# Autodesk Inventor assembly: Scananlage_Adrian
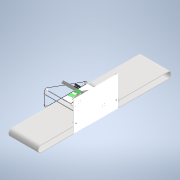
[picture p0: Inventor's stored thumbnail of the model, 180x180]
Saved by Autodesk Inventor 2021 (Build 250183000, 183)
## iProperties
Created: 2022-07-12
Part Number: Scananlage_Adrian
Document SubType Name: Assembly
Designer: adria
Mass: 34959.8 g
Surface Area: 77259.1 cm^2
Volume: 43992.2 cm^3
Density: 0.794683 g/cm^3
Author: adria
## Documents named in this file (16)
- C:\Users\adria\OneDrive - tum.de\G2_Waste-Recycling\CAD\Scananlage_Adrian.iam
- C:\Users\adria\OneDrive - tum.de\G2_Waste-Recycling\CAD\Adrian_Box.iam
- C:\Users\adria\OneDrive - tum.de\G2_Waste-Recycling\CAD\Adrian_Stangeantrieb.iam
- C:\Users\adria\OneDrive - tum.de\G2_Waste-Recycling\CAD\Adrian_Rolle.iam
- C:\Users\adria\OneDrive - tum.de\G2_Waste-Recycling\CAD\stepper-motor-nema17-simplified-model-1.snapshot.3\motor.ipt
- C:\Users\adria\OneDrive - tum.de\G2_Waste-Recycling\CAD\Adrian_Drehteller.iam
- C:\Users\adria\OneDrive - tum.de\G2_Waste-Recycling\CAD\Adrian_Cameraarm.iam
- C:\Users\adria\OneDrive - tum.de\G2_Waste-Recycling\CAD\Adrian_Faden.ipt
- C:\Users\adria\OneDrive - tum.de\G2_Waste-Recycling\CAD\Stange_SCHIEBER.ipt
- C:\Users\adria\OneDrive - tum.de\G2_Waste-Recycling\CAD\GT2 Timing Pulley T40.ipt
- C:\Users\adria\OneDrive - tum.de\G2_Waste-Recycling\CAD\Adrian_Riemen.ipt
- C:\Users\adria\OneDrive - tum.de\G2_Waste-Recycling\CAD\Assembly Raspberry Pi 4 Model B step.ipt
- C:\Users\adria\OneDrive - tum.de\G2_Waste-Recycling\CAD\Ethernet SmoothStepper_ASSEMBLY.ipt
- C:\Users\adria\Documents\Inventor\Content Center Files\R2021\de-DE\ISO 1207(2)\ISO 1207 - M2 x 6.ipt
- C:\Users\adria\Documents\Inventor\Content Center Files\R2021\de-DE\ISO 4762(2)\ISO 4762 - M3 x 30ISO.ipt
- C:\Users\adria\OneDrive - tum.de\G2_Waste-Recycling\CAD\Adrian_Förderband.ipt
## Components (35 placed, 15 different names)
1. Adrian_Box:1 [sub-assembly] — Passend:1, Fluchtend:1, Passend:2, Passend:3, Passend:4, Passend:5, Passend:6, Passend:7, Passend:8, Passend:9, Passend:10, Passend:11, Passend:12, Passend:13, Passend:14, Passend:15, Passend:16, Passend:17, Passend:18, Passend:19, Passend:24, Passend:25, Passend:32, Fluchtend:3, Passend:33, Passend:34, Fluchtend:4, Passend:44, Passend:45, Passend:46, Passend:47, Passend:48, Passend:49, Passend:50, Passend:51, Passend:52, Passend:53, Passend:54, Passend:55, Passend:56, Passend:57, Passend:58, Passend:59, Passend:60, Passend:61, Passend:62, Passend:63, Passend:64, Passend:65, Passend:66, Passend:67, Fluchtend:6, Fluchtend:7, Fluchtend:10
2. Adrian_Stangeantrieb:1 [sub-assembly] — Passend:1, Fluchtend:1, Passend:31
3. Adrian_Rolle:1 [sub-assembly] — Passend:2, Passend:3
4. Adrian_Rolle:2 [sub-assembly] — Passend:6, Passend:9, Passend:23
5. Adrian_Rolle:3 [sub-assembly] — Passend:5, Passend:8, Passend:22
6. Adrian_Rolle:4 [sub-assembly] — Passend:4, Passend:7, Passend:26, Passend:27
7. motor:1 — Passend:10, Passend:11, Passend:16, Passend:28, Passend:29, Winkel:1, Fluchtend:2
8. motor:3 — Passend:12, Passend:13, Passend:14, Passend:15, Passend:20, Passend:21
9. Adrian_Drehteller:1 [sub-assembly] — Passend:17, Passend:18, Passend:19
10. Adrian_Cameraarm:1 [sub-assembly] — Passend:20, Passend:21
11. Adrian_Faden:1 — Passend:22, Passend:24, Passend:27, Tangential:1
12. Adrian_Faden:2 — Passend:23, Passend:25
13. Stange_SCHIEBER:1 — Passend:26, Tangential:1
14. GT2 Timing Pulley T40:1 — Passend:28, Passend:29, Passend:30
15. Adrian_Riemen:1 — Winkel:1, Passend:30, Passend:31, Fluchtend:2
16. Assembly Raspberry Pi 4 Model B step:1 — Passend:32, Fluchtend:3, Passend:33, Passend:35, Passend:38, Passend:39, Passend:40, Passend:41
17. Ethernet SmoothStepper_ASSEMBLY:1 — Passend:34, Fluchtend:4, Passend:35, Passend:36, Passend:37, Passend:42, Passend:43
18. ISO 1207 M2 x 6:1 — Passend:37, Passend:43
19. ISO 1207 M2 x 6:2 — Passend:36, Passend:42
20. ISO 1207 M2 x 6:3 — Passend:39, Passend:40
21. ISO 1207 M2 x 6:4 — Passend:38, Passend:41
22. ISO 4762 M3 x 30:3 — Passend:46, Passend:49
23. ISO 4762 M3 x 30:4 — Passend:44, Passend:51
24. ISO 4762 M3 x 30:5 — Passend:47, Passend:50
25. ISO 4762 M3 x 30:6 — Passend:45, Passend:48
26. ISO 4762 M3 x 30:7 — Passend:52, Passend:58
27. ISO 4762 M3 x 30:8 — Passend:55, Passend:56
28. ISO 4762 M3 x 30:9 — Passend:53, Passend:59
29. ISO 4762 M3 x 30:10 — Passend:54, Passend:57
30. ISO 4762 M3 x 30:11 — Passend:61, Passend:65
31. ISO 4762 M3 x 30:12 — Passend:60, Passend:67
32. ISO 4762 M3 x 30:13 — Passend:63, Passend:64
33. ISO 4762 M3 x 30:14 — Passend:62, Passend:66
34. Adrian_Förderband:1 — Fluchtend:5, Fluchtend:6, Fluchtend:7, Fluchtend:8
35. Adrian_Förderband:2 — Fluchtend:5, Fluchtend:8
## Relationships (78: Mate 67, Flush 9, Tangent 1, Angle 1)
- Passend:1 [Mate]: Adrian_Box:1 ↔ Adrian_Stangeantrieb:1
- Fluchtend:1 [Flush]: Adrian_Box:1 ↔ Adrian_Stangeantrieb:1
- Passend:2 [Mate]: Adrian_Box:1 ↔ Adrian_Rolle:1
- Passend:3 [Mate]: Adrian_Box:1 ↔ Adrian_Rolle:1
- Passend:4 [Mate]: Adrian_Box:1 ↔ Adrian_Rolle:4
- Passend:5 [Mate]: Adrian_Box:1 ↔ Adrian_Rolle:3
- Passend:6 [Mate]: Adrian_Box:1 ↔ Adrian_Rolle:2
- Passend:7 [Mate]: Adrian_Box:1 ↔ Adrian_Rolle:4
- Passend:8 [Mate]: Adrian_Box:1 ↔ Adrian_Rolle:3
- Passend:9 [Mate]: Adrian_Box:1 ↔ Adrian_Rolle:2
- Passend:10 [Mate]: Adrian_Box:1 ↔ motor:1
- Passend:11 [Mate]: Adrian_Box:1 ↔ motor:1
- Passend:12 [Mate]: Adrian_Box:1 ↔ motor:3
- Passend:13 [Mate]: Adrian_Box:1 ↔ motor:3
- Passend:14 [Mate]: Adrian_Box:1 ↔ motor:3
- Passend:15 [Mate]: Adrian_Box:1 ↔ motor:3
- Passend:16 [Mate]: Adrian_Box:1 ↔ motor:1
- Passend:17 [Mate]: Adrian_Box:1 ↔ Adrian_Drehteller:1
- Passend:18 [Mate]: Adrian_Box:1 ↔ Adrian_Drehteller:1
- Passend:19 [Mate]: Adrian_Box:1 ↔ Adrian_Drehteller:1
- Passend:20 [Mate]: motor:3 ↔ Adrian_Cameraarm:1
- Passend:21 [Mate]: motor:3 ↔ Adrian_Cameraarm:1
- Passend:22 [Mate]: Adrian_Rolle:3 ↔ Adrian_Faden:1
- Passend:23 [Mate]: Adrian_Rolle:2 ↔ Adrian_Faden:2
- Passend:24 [Mate] (10 mm): Adrian_Box:1 ↔ Adrian_Faden:1
- Passend:25 [Mate] (10 mm): Adrian_Box:1 ↔ Adrian_Faden:2
- Passend:26 [Mate]: Adrian_Rolle:4 ↔ Stange_SCHIEBER:1
- Passend:27 [Mate]: Adrian_Rolle:4 ↔ Adrian_Faden:1
- Tangential:1: Adrian_Faden:1 ↔ Stange_SCHIEBER:1
- Passend:28 [Mate]: motor:1 ↔ GT2 Timing Pulley T40:1
- Passend:29 [Mate]: motor:1 ↔ GT2 Timing Pulley T40:1
- Winkel:1 [Angle] (0 deg): motor:1 ↔ Adrian_Riemen:1
- Passend:30 [Mate]: GT2 Timing Pulley T40:1 ↔ Adrian_Riemen:1
- Passend:31 [Mate]: Adrian_Stangeantrieb:1 ↔ Adrian_Riemen:1
- Fluchtend:2 [Flush] (-7 mm): motor:1 ↔ Adrian_Riemen:1
- Passend:32 [Mate]: Adrian_Box:1 ↔ Assembly Raspberry Pi 4 Model B step:1
- Fluchtend:3 [Flush] (40 mm): Adrian_Box:1 ↔ Assembly Raspberry Pi 4 Model B step:1
- Passend:33 [Mate] (40 mm): Adrian_Box:1 ↔ Assembly Raspberry Pi 4 Model B step:1
- Passend:34 [Mate]: Adrian_Box:1 ↔ Ethernet SmoothStepper_ASSEMBLY:1
- Fluchtend:4 [Flush] (40 mm): Adrian_Box:1 ↔ Ethernet SmoothStepper_ASSEMBLY:1
- Passend:35 [Mate] (40 mm): Assembly Raspberry Pi 4 Model B step:1 ↔ Ethernet SmoothStepper_ASSEMBLY:1
- Passend:36 [Mate]: Ethernet SmoothStepper_ASSEMBLY:1 ↔ ISO 1207 M2 x 6:2
- Passend:37 [Mate]: Ethernet SmoothStepper_ASSEMBLY:1 ↔ ISO 1207 M2 x 6:1
- Passend:38 [Mate]: Assembly Raspberry Pi 4 Model B step:1 ↔ ISO 1207 M2 x 6:4
- Passend:39 [Mate]: Assembly Raspberry Pi 4 Model B step:1 ↔ ISO 1207 M2 x 6:3
- Passend:40 [Mate]: Assembly Raspberry Pi 4 Model B step:1 ↔ ISO 1207 M2 x 6:3
- Passend:41 [Mate]: Assembly Raspberry Pi 4 Model B step:1 ↔ ISO 1207 M2 x 6:4
- Passend:42 [Mate]: Ethernet SmoothStepper_ASSEMBLY:1 ↔ ISO 1207 M2 x 6:2
- Passend:43 [Mate]: Ethernet SmoothStepper_ASSEMBLY:1 ↔ ISO 1207 M2 x 6:1
- Passend:44 [Mate]: Adrian_Box:1 ↔ ISO 4762 M3 x 30:4
- Passend:45 [Mate]: Adrian_Box:1 ↔ ISO 4762 M3 x 30:6
- Passend:46 [Mate]: Adrian_Box:1 ↔ ISO 4762 M3 x 30:3
- Passend:47 [Mate]: Adrian_Box:1 ↔ ISO 4762 M3 x 30:5
- Passend:48 [Mate]: Adrian_Box:1 ↔ ISO 4762 M3 x 30:6
- Passend:49 [Mate]: Adrian_Box:1 ↔ ISO 4762 M3 x 30:3
- Passend:50 [Mate]: Adrian_Box:1 ↔ ISO 4762 M3 x 30:5
- Passend:51 [Mate]: Adrian_Box:1 ↔ ISO 4762 M3 x 30:4
- Passend:52 [Mate]: Adrian_Box:1 ↔ ISO 4762 M3 x 30:7
- Passend:53 [Mate]: Adrian_Box:1 ↔ ISO 4762 M3 x 30:9
- Passend:54 [Mate]: Adrian_Box:1 ↔ ISO 4762 M3 x 30:10
- Passend:55 [Mate]: Adrian_Box:1 ↔ ISO 4762 M3 x 30:8
- Passend:56 [Mate]: Adrian_Box:1 ↔ ISO 4762 M3 x 30:8
- Passend:57 [Mate]: Adrian_Box:1 ↔ ISO 4762 M3 x 30:10
- Passend:58 [Mate]: Adrian_Box:1 ↔ ISO 4762 M3 x 30:7
- Passend:59 [Mate]: Adrian_Box:1 ↔ ISO 4762 M3 x 30:9
- Passend:60 [Mate]: Adrian_Box:1 ↔ ISO 4762 M3 x 30:12
- Passend:61 [Mate]: Adrian_Box:1 ↔ ISO 4762 M3 x 30:11
- Passend:62 [Mate]: Adrian_Box:1 ↔ ISO 4762 M3 x 30:14
- Passend:63 [Mate]: Adrian_Box:1 ↔ ISO 4762 M3 x 30:13
- Passend:64 [Mate]: Adrian_Box:1 ↔ ISO 4762 M3 x 30:13
- Passend:65 [Mate]: Adrian_Box:1 ↔ ISO 4762 M3 x 30:11
- Passend:66 [Mate]: Adrian_Box:1 ↔ ISO 4762 M3 x 30:14
- Passend:67 [Mate]: Adrian_Box:1 ↔ ISO 4762 M3 x 30:12
- Fluchtend:5 [Flush]: Adrian_Förderband:1 ↔ Adrian_Förderband:2
- Fluchtend:6 [Flush]: Adrian_Box:1 ↔ Adrian_Förderband:1
- Fluchtend:7 [Flush]: Adrian_Box:1 ↔ Adrian_Förderband:1
- Fluchtend:8 [Flush]: Adrian_Förderband:1 ↔ Adrian_Förderband:2
- Fluchtend:10 [Flush] (600 mm): Adrian_Box:1
